# Autodesk Inventor assembly: Gearbox
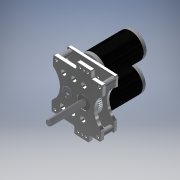
[picture p0: Inventor's stored thumbnail of the model, 180x180]
Saved by Autodesk Inventor 2019 (Build 230136000, 136)
## iProperties
Created: 2018-01-18
Part Number: Gearbox
Document SubType Name: Assembly
Designer: maste
Author: maste
## Documents named in this file (13)
- D:\Summer Drive Base V1\Summer Drivebase\Gearbox.iam
- D:\Summer Drive Base V1\Summer Drivebase\Drivebase PowerUp Files\new_folder__2_\New folder (2)\am-2725+3CIM4U+Motor+Plate+r2.ipt
- D:\Summer Drive Base V1\Summer Drivebase\Drivebase PowerUp Files\am-2035+45+Tooth+Aluminum+Gear+with+500+Hex+Bore.ipt
- D:\Summer Drive Base V1\Summer Drivebase\Drivebase PowerUp Files\14t_Steel_Spur_Gear_20_DP_CIM_Motor_217-3414.ipt
- D:\Summer Drive Base V1\Summer Drivebase\Drivebase PowerUp Files\CIM_Motor_217-2000.ipt
- D:\Summer Drive Base V1\Summer Drivebase\Drivebase PowerUp Files\FR6ZZ Bearing Copy.ipt
- D:\Summer Drive Base V1\Summer Drivebase\Drivebase PowerUp Files\Not Tiberculosis TB Hex Shaft.ipt
- D:\Summer Drive Base V1\Summer Drivebase\Drivebase PowerUp Files\am-0149+Toughbox+Large+Cluster+Gear.ipt
- D:\Summer Drive Base V1\Summer Drivebase\Drivebase PowerUp Files\am-0176_19T20dp375h.ipt
- D:\Summer Drive Base V1\Summer Drivebase\Drivebase PowerUp Files\Not Tiberculosis TB Output Shaft Hex L-Base 2.ipt
- D:\Summer Drive Base V1\Summer Drivebase\Drivebase PowerUp Files\2nd Plate.ipt
- D:\Summer Drive Base V1\Summer Drivebase\Drivebase PowerUp Files\0_500_Hex_ID_x_1_125_OD_x_0_313_WD_Flanged_Bearing_v2_217-3875.ipt
- D:\Summer Drive Base V1\Summer Drivebase\Drivebase PowerUp Files\Pretend this is a churro.ipt
## Components (19 placed, 12 different names)
1. am-2725+3CIM4U+Motor+Plate+r2:1 — Mate:5, Mate:6, Mate:7, Mate:8, Mate:9, Mate:10, Mate:12, Mate:13, Rotation:3, Mate:14, Mate:15, Rotation:4, Mate:37, Mate:43, Mate:44, Mate:45
2. am-2035+45+Tooth+Aluminum+Gear+with+500+Hex+Bore:1 — Mate:27, Mate:28, Mate:29
3. 14t_Steel_Spur_Gear_20_DP_CIM_Motor_217-3414:1 — Mate:1, Mate:2, Rotation:1
4. 14t_Steel_Spur_Gear_20_DP_CIM_Motor_217-3414:2 — Mate:3, Mate:4, Rotation:2
5. CIM_Motor_217-2000:1 — Mate:3, Mate:4, Rotation:2, Mate:5, Mate:6, Mate:10
6. CIM_Motor_217-2000:2 — Mate:1, Mate:2, Rotation:1, Mate:7, Mate:8, Mate:9
7. FR6ZZ Bearing Copy:1 — Mate:14, Mate:15, Rotation:4, Mate:25, Mate:26, Rotation:7
8. FR6ZZ Bearing Copy:2 — Mate:12, Mate:13, Rotation:3, Mate:17, Mate:18, Rotation:5, Mate:19
9. Not Tiberculosis TB Hex Shaft:1 — Mate:17, Mate:18, Rotation:5, Mate:20, Mate:21, Rotation:6, Mate:23, Mate:24, Rotation:11
10. am-0149+Toughbox+Large+Cluster+Gear:1 — Mate:19, Mate:20, Mate:21, Rotation:6, Mate:22
11. am-0176_19T20dp375h:1 — Mate:22, Mate:23, Mate:24
12. Not Tiberculosis TB Output Shaft Hex L-Base 2:1 — Mate:25, Mate:26, Rotation:7, Mate:27, Mate:28, Mate:29, Mate:36
13. 2nd Plate:1 — Mate:33, Rotation:10, Mate:39, Mate:41, Mate:42, Mate:46, Mate:47, Mate:48
14. FR6ZZ Bearing Copy:3 — Rotation:11, Mate:48
15. 0_500_Hex_ID_x_1_125_OD_x_0_313_WD_Flanged_Bearing_v2_217-3875:1 — Mate:33, Rotation:10, Mate:36
16. Pretend this is a churro:1 — Mate:44, Mate:45
17. Pretend this is a churro:2 — Mate:37, Mate:39
18. Pretend this is a churro:3 — Mate:41, Mate:42, Mate:46
19. Pretend this is a churro:4 — Mate:43, Mate:47
## Relationships (48: Mate 39, RelateRotation 9)
- Mate:1: 14t_Steel_Spur_Gear_20_DP_CIM_Motor_217-3414:1 ↔ CIM_Motor_217-2000:2
- Mate:2: 14t_Steel_Spur_Gear_20_DP_CIM_Motor_217-3414:1 ↔ CIM_Motor_217-2000:2
- Rotation:1 [RelateRotation] (1 ul): 14t_Steel_Spur_Gear_20_DP_CIM_Motor_217-3414:1 ↔ CIM_Motor_217-2000:2
- Mate:3: 14t_Steel_Spur_Gear_20_DP_CIM_Motor_217-3414:2 ↔ CIM_Motor_217-2000:1
- Mate:4: 14t_Steel_Spur_Gear_20_DP_CIM_Motor_217-3414:2 ↔ CIM_Motor_217-2000:1
- Rotation:2 [RelateRotation] (1 ul): 14t_Steel_Spur_Gear_20_DP_CIM_Motor_217-3414:2 ↔ CIM_Motor_217-2000:1
- Mate:5: am-2725+3CIM4U+Motor+Plate+r2:1 ↔ CIM_Motor_217-2000:1
- Mate:6: am-2725+3CIM4U+Motor+Plate+r2:1 ↔ CIM_Motor_217-2000:1
- Mate:7: am-2725+3CIM4U+Motor+Plate+r2:1 ↔ CIM_Motor_217-2000:2
- Mate:8: am-2725+3CIM4U+Motor+Plate+r2:1 ↔ CIM_Motor_217-2000:2
- Mate:9: am-2725+3CIM4U+Motor+Plate+r2:1 ↔ CIM_Motor_217-2000:2
- Mate:10: am-2725+3CIM4U+Motor+Plate+r2:1 ↔ CIM_Motor_217-2000:1
- Mate:12: am-2725+3CIM4U+Motor+Plate+r2:1 ↔ FR6ZZ Bearing Copy:2
- Mate:13: am-2725+3CIM4U+Motor+Plate+r2:1 ↔ FR6ZZ Bearing Copy:2
- Rotation:3 [RelateRotation] (1 ul): am-2725+3CIM4U+Motor+Plate+r2:1 ↔ FR6ZZ Bearing Copy:2
- Mate:14: am-2725+3CIM4U+Motor+Plate+r2:1 ↔ FR6ZZ Bearing Copy:1
- Mate:15: am-2725+3CIM4U+Motor+Plate+r2:1 ↔ FR6ZZ Bearing Copy:1
- Rotation:4 [RelateRotation] (1 ul): am-2725+3CIM4U+Motor+Plate+r2:1 ↔ FR6ZZ Bearing Copy:1
- Mate:17: FR6ZZ Bearing Copy:2 ↔ Not Tiberculosis TB Hex Shaft:1
- Mate:18: FR6ZZ Bearing Copy:2 ↔ Not Tiberculosis TB Hex Shaft:1
- Rotation:5 [RelateRotation] (1 ul): FR6ZZ Bearing Copy:2 ↔ Not Tiberculosis TB Hex Shaft:1
- Mate:19: FR6ZZ Bearing Copy:2 ↔ am-0149+Toughbox+Large+Cluster+Gear:1
- Mate:20: Not Tiberculosis TB Hex Shaft:1 ↔ am-0149+Toughbox+Large+Cluster+Gear:1
- Mate:21: Not Tiberculosis TB Hex Shaft:1 ↔ am-0149+Toughbox+Large+Cluster+Gear:1
- Rotation:6 [RelateRotation] (1 ul): Not Tiberculosis TB Hex Shaft:1 ↔ am-0149+Toughbox+Large+Cluster+Gear:1
- Mate:22: am-0149+Toughbox+Large+Cluster+Gear:1 ↔ am-0176_19T20dp375h:1
- Mate:23: Not Tiberculosis TB Hex Shaft:1 ↔ am-0176_19T20dp375h:1
- Mate:24: Not Tiberculosis TB Hex Shaft:1 ↔ am-0176_19T20dp375h:1
- Mate:25: FR6ZZ Bearing Copy:1 ↔ Not Tiberculosis TB Output Shaft Hex L-Base 2:1
- Mate:26: FR6ZZ Bearing Copy:1 ↔ Not Tiberculosis TB Output Shaft Hex L-Base 2:1
- Rotation:7 [RelateRotation] (1 ul): FR6ZZ Bearing Copy:1 ↔ Not Tiberculosis TB Output Shaft Hex L-Base 2:1
- Mate:27: am-2035+45+Tooth+Aluminum+Gear+with+500+Hex+Bore:1 ↔ Not Tiberculosis TB Output Shaft Hex L-Base 2:1
- Mate:28: am-2035+45+Tooth+Aluminum+Gear+with+500+Hex+Bore:1 ↔ Not Tiberculosis TB Output Shaft Hex L-Base 2:1
- Mate:29: am-2035+45+Tooth+Aluminum+Gear+with+500+Hex+Bore:1 ↔ Not Tiberculosis TB Output Shaft Hex L-Base 2:1
- Mate:33: 2nd Plate:1 ↔ 0_500_Hex_ID_x_1_125_OD_x_0_313_WD_Flanged_Bearing_v2_217-3875:1
- Rotation:10 [RelateRotation] (1 ul): 2nd Plate:1 ↔ 0_500_Hex_ID_x_1_125_OD_x_0_313_WD_Flanged_Bearing_v2_217-3875:1
- Mate:36: Not Tiberculosis TB Output Shaft Hex L-Base 2:1 ↔ 0_500_Hex_ID_x_1_125_OD_x_0_313_WD_Flanged_Bearing_v2_217-3875:1
- Mate:37: am-2725+3CIM4U+Motor+Plate+r2:1 ↔ Pretend this is a churro:2
- Mate:39: 2nd Plate:1 ↔ Pretend this is a churro:2
- Mate:41: 2nd Plate:1 ↔ Pretend this is a churro:3
- Mate:42: 2nd Plate:1 ↔ Pretend this is a churro:3
- Mate:43: am-2725+3CIM4U+Motor+Plate+r2:1 ↔ Pretend this is a churro:4
- Mate:44: am-2725+3CIM4U+Motor+Plate+r2:1 ↔ Pretend this is a churro:1
- Mate:45: am-2725+3CIM4U+Motor+Plate+r2:1 ↔ Pretend this is a churro:1
- Mate:46: 2nd Plate:1 ↔ Pretend this is a churro:3
- Mate:47: 2nd Plate:1 ↔ Pretend this is a churro:4
- Rotation:11 [RelateRotation] (1.003 ul): Not Tiberculosis TB Hex Shaft:1 ↔ FR6ZZ Bearing Copy:3
- Mate:48: 2nd Plate:1 ↔ FR6ZZ Bearing Copy:3
